# Autodesk Inventor assembly: ROBOT_5GDL
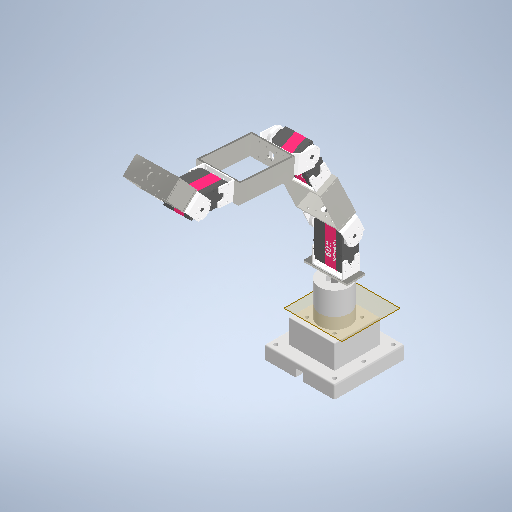
[picture p0: Inventor's stored thumbnail of the model, 512x512]
Saved by Autodesk Inventor 2025.1 (Build 291241000, 241)
## iProperties
Created: 2024-12-02
Part Number: ROBOT_5GDL
Document SubType Name: Assembly
Designer: Cristhian Vigo
Author: Cristhian Vigo
## Documents named in this file (15)
- D:\CRISTHIAN\universidad\ciclo 8\Robótica\PROYECTO\Modelo\ROBOT_5GDL\ROBOT_5GDL Movimiento.iam
- D:\CRISTHIAN\universidad\ciclo 8\Robótica\PROYECTO\Modelo\ROBOT_5GDL\base.ipt
- D:\CRISTHIAN\universidad\ciclo 8\Robótica\PROYECTO\Modelo\ROBOT_5GDL\Servo.ipt
- D:\CRISTHIAN\universidad\ciclo 8\Robótica\PROYECTO\Modelo\ROBOT_5GDL\base giratoria.ipt
- D:\CRISTHIAN\universidad\ciclo 8\Robótica\PROYECTO\Modelo\ROBOT_5GDL\engranaje recto servo.ipt
- D:\CRISTHIAN\universidad\ciclo 8\Robótica\PROYECTO\Modelo\ROBOT_5GDL\rodamiento.ipt
- D:\CRISTHIAN\universidad\ciclo 8\Robótica\PROYECTO\Modelo\ROBOT_5GDL\Soporte 1.ipt
- D:\CRISTHIAN\universidad\ciclo 8\Robótica\PROYECTO\Modelo\ROBOT_5GDL\Soporte 2.ipt
- D:\CRISTHIAN\universidad\ciclo 8\Robótica\PROYECTO\Modelo\ROBOT_5GDL\Eslabón3.iam
- D:\CRISTHIAN\universidad\ciclo 8\Robótica\PROYECTO\Modelo\ROBOT_5GDL\Eslabón4.iam
- D:\CRISTHIAN\universidad\ciclo 8\Robótica\PROYECTO\Modelo\ROBOT_5GDL\NEMA 23 - 41mm\Inventor\NEMA 23 - 41mm.iam
- D:\CRISTHIAN\universidad\ciclo 8\Robótica\PROYECTO\Modelo\ROBOT_5GDL\Eslabón2.iam
- D:\CRISTHIAN\universidad\ciclo 8\Robótica\PROYECTO\Modelo\ROBOT_5GDL\Base_eslabón.ipt
- D:\CRISTHIAN\universidad\ciclo 8\Robótica\PROYECTO\Modelo\ROBOT_5GDL\Eslabon1.ipt
- D:\CRISTHIAN\universidad\ciclo 8\Robótica\PROYECTO\Modelo\ROBOT_5GDL\Eje8mm.ipt
## Components (28 placed, 14 different names)
1. base:1
2. Servo:1
3. base giratoria:1
4. engranaje recto servo:1
5. rodamiento:1
6. Soporte 1:1 — Flush:1, Flush:2, Mate:7
7. Soporte 2:1 — Flush:7, Flush:8, Mate:16
8. Eslabón3:1 [sub-assembly] — Flush:1, Flush:2, Mate:7, Mate:14, Flush:3, Flush:4
9. base:2
10. Servo:2
11. base giratoria:2
12. engranaje recto servo:2
13. rodamiento:2
14. Soporte 1:2 — Flush:5, Flush:6, Mate:15
15. Soporte 2:2 — Mate:14, Flush:3, Flush:4
16. Eslabón4:1 [sub-assembly] — Flush:5, Flush:6, Mate:15
17. NEMA 23 - 41mm:1 [sub-assembly] — Insert:106, Insert:107
18. Eslabón2:1 [sub-assembly] — Flush:7, Flush:8, Mate:16, Flush:9, Flush:10, Mate:23
19. base:3
20. Servo:3
21. base giratoria:3
22. engranaje recto servo:3
23. rodamiento:3
24. Soporte 1:3 — Flush:9, Flush:10, Mate:23, Flush:13
25. Soporte 2:3 — Mate:25, Flush:14
26. Base_eslabón:1 — Mate:25, Flush:13, Flush:14, Insert:108
27. Eslabon1:1 — Insert:106, Insert:107, Insert:109
28. Eje8mm:1 — Insert:108, Insert:109
## Relationships (52: Mate 24, Insert 16, Flush 12)
- [Mate]: Servo:1 ↔ Soporte 2:1
- [Mate]: Servo:1 ↔ Soporte 2:1
- [Mate]: Servo:1 ↔ Soporte 2:1
- [Insert]: base:1 ↔ rodamiento:1
- [Insert]: base:1 ↔ Servo:1
- [Insert]: Servo:1 ↔ engranaje recto servo:1
- [Insert]: base giratoria:1 ↔ engranaje recto servo:1
- [Mate]: base giratoria:1 ↔ Soporte 1:1
- [Mate]: base giratoria:1 ↔ Soporte 1:1
- [Mate]: base:1 ↔ Soporte 1:1
- Flush:1: Soporte 1:1 ↔ Eslabón3:1
- Flush:2 (-1 mm): Soporte 1:1 ↔ Eslabón3:1
- Mate:7: Soporte 1:1 ↔ Eslabón3:1
- [Mate]: Servo:2 ↔ Soporte 2:2
- [Mate]: Servo:2 ↔ Soporte 2:2
- [Mate]: Servo:2 ↔ Soporte 2:2
- [Insert]: base:2 ↔ rodamiento:2
- [Insert]: base:2 ↔ Servo:2
- [Insert]: Servo:2 ↔ engranaje recto servo:2
- [Insert]: base giratoria:2 ↔ engranaje recto servo:2
- [Mate]: base giratoria:2 ↔ Soporte 1:2
- [Mate]: base giratoria:2 ↔ Soporte 1:2
- [Mate]: base:2 ↔ Soporte 1:2
- Mate:14: Eslabón3:1 ↔ Soporte 2:2
- Flush:3 (-1 mm): Eslabón3:1 ↔ Soporte 2:2
- Flush:4 (8 mm): Eslabón3:1 ↔ Soporte 2:2
- Flush:5: Soporte 1:2 ↔ Eslabón4:1
- Flush:6 (-1 mm): Soporte 1:2 ↔ Eslabón4:1
- Mate:15: Soporte 1:2 ↔ Eslabón4:1
- Flush:7 (8 mm): Soporte 2:1 ↔ Eslabón2:1
- Flush:8 (-1 mm): Soporte 2:1 ↔ Eslabón2:1
- Mate:16: Soporte 2:1 ↔ Eslabón2:1
- [Mate]: Servo:3 ↔ Soporte 2:3
- [Mate]: Servo:3 ↔ Soporte 2:3
- [Mate]: Servo:3 ↔ Soporte 2:3
- [Insert]: base:3 ↔ rodamiento:3
- [Insert]: base:3 ↔ Servo:3
- [Insert]: Servo:3 ↔ engranaje recto servo:3
- [Insert]: base giratoria:3 ↔ engranaje recto servo:3
- [Mate]: base giratoria:3 ↔ Soporte 1:3
- [Mate]: base giratoria:3 ↔ Soporte 1:3
- [Mate]: base:3 ↔ Soporte 1:3
- Flush:9: Eslabón2:1 ↔ Soporte 1:3
- Flush:10 (-1 mm): Eslabón2:1 ↔ Soporte 1:3
- Mate:23: Eslabón2:1 ↔ Soporte 1:3
- Mate:25: Soporte 2:3 ↔ Base_eslabón:1
- Flush:13: Soporte 1:3 ↔ Base_eslabón:1
- Flush:14 (-1 mm): Soporte 2:3 ↔ Base_eslabón:1
- Insert:106: NEMA 23 - 41mm:1 ↔ Eslabon1:1
- Insert:107: NEMA 23 - 41mm:1 ↔ Eslabon1:1
- Insert:108: Base_eslabón:1 ↔ Eje8mm:1
- Insert:109 (-28 mm): Eslabon1:1 ↔ Eje8mm:1
## Named parameters: d0_d4 = 0 mm, d1_d5 = 0 mm, d2_d6 = 0 mm, d16_d25 = 0 mm, d17_d26 = 0 mm, d56_d0_d4 = 0 mm, d57_d1_d5 = 0 mm, d58_d2_d6 = 0 mm, d70_d14 = 0 mm, d71_d15 = 0 mm, d72_d16_d25 = 0 mm, d73_d17_d26 = 0 mm, d78_d31 = 0 mm, d79_d32 = 0 mm, d80_d33 = 0 mm, d95_d0_d4 = 0 mm, d96_d1_d5 = 0 mm, d97_d2_d6 = 0 mm, d109_d14 = 0 mm, d110_d15 = 0 mm, d111_d16_d25 = 0 mm, d112_d17_d26 = 0 mm, d117_d31 = 0 mm, d118_d32 = 0 mm, d119_d33 = 0 mm
